# Autodesk Inventor assembly: Differential Swerve Drive V3
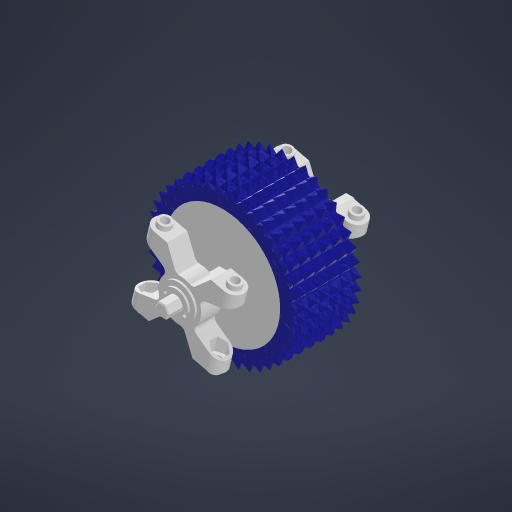
[picture p0: Inventor's stored thumbnail of the model, 512x512]
Saved by Autodesk Inventor 2024 (Build 280153000, 153)
## iProperties
Created: 2023-09-09
Part Number: Differential Swerve Drive V3
Document SubType Name: Assembly
Designer: izack
Author: izack
## Documents named in this file (7)
- C:\Users\izack\Robotics\CAD\Custom-Modules-CAD\Differential Swerve Drive V1\Differential Swerve Drive V3.iam
- C:\Users\izack\Robotics\CAD\Custom-Modules-CAD\Differential Swerve Drive V1\Differential Swerve Drive V3\60mm Wheel Rim.ipt
- C:\Users\izack\Robotics\CAD\Custom-Modules-CAD\Differential Swerve Drive V1\Differential Swerve Drive V3\60mm Wheel Tire Tread.ipt
- C:\Users\izack\Robotics\CAD\Custom-Modules-CAD\Differential Swerve Drive V1\Differential Swerve Drive V3\5mm x 55mm Hex Shaft.ipt
- C:\Users\izack\Robotics\CAD\Custom-Modules-CAD\Differential Swerve Drive V1\Differential Swerve Drive V3\Center_Bracket.ipt
- C:\Users\izack\Robotics\CAD\Custom-Modules-CAD\Differential Swerve Drive V1\Differential Swerve Drive V3\Flanged_Bearing.ipt
- C:\Users\izack\Robotics\CAD\Custom-Modules-CAD\Differential Swerve Drive V1\Differential Swerve Drive V3\5mm Hex to 8mm Round Bearing Insert.ipt
## Components (13 placed, 6 different names)
1. 60mm Wheel Rim:1 — Flush:1, Mate:1, Mate:2
2. 60mm Wheel Tire Tread:1 — Flush:1
3. 5mm x 55mm Hex Shaft:1 — Mate:1, Mate:2, Mate:19, Mate:20, Mate:21, Mate:23, Mate:24
4. Center_Bracket:1 — Mate:5, Mate:6, Mate:13, Mate:14, Flush:2
5. Center_Bracket:2 — Mate:15, Mate:16, Mate:17, Mate:18, Mate:22, Flush:2
6. Flanged_Bearing:1 — Mate:11, Mate:12, Mate:17, Mate:18
7. Flanged_Bearing:2 — Mate:9, Mate:10, Mate:15, Mate:16, Mate:22
8. Flanged_Bearing:3 — Mate:3, Mate:4, Mate:5, Mate:6
9. Flanged_Bearing:4 — Mate:7, Mate:8, Mate:13, Mate:14
10. 5mm Hex to 8mm Round Bearing Insert:1 — Mate:11, Mate:12, Mate:21, Mate:23
11. 5mm Hex to 8mm Round Bearing Insert:2 — Mate:9, Mate:10, Mate:24
12. 5mm Hex to 8mm Round Bearing Insert:3 — Mate:7, Mate:8
13. 5mm Hex to 8mm Round Bearing Insert:4 — Mate:3, Mate:4, Mate:19, Mate:20
## Relationships (26: Mate 24, Flush 2)
- Flush:1: 60mm Wheel Rim:1 ↔ 60mm Wheel Tire Tread:1
- Mate:1: 60mm Wheel Rim:1 ↔ 5mm x 55mm Hex Shaft:1
- Mate:2: 60mm Wheel Rim:1 ↔ 5mm x 55mm Hex Shaft:1
- Mate:3: Flanged_Bearing:3 ↔ 5mm Hex to 8mm Round Bearing Insert:4
- Mate:4: Flanged_Bearing:3 ↔ 5mm Hex to 8mm Round Bearing Insert:4
- Mate:5: Center_Bracket:1 ↔ Flanged_Bearing:3
- Mate:6: Center_Bracket:1 ↔ Flanged_Bearing:3
- Mate:7: Flanged_Bearing:4 ↔ 5mm Hex to 8mm Round Bearing Insert:3
- Mate:8: Flanged_Bearing:4 ↔ 5mm Hex to 8mm Round Bearing Insert:3
- Mate:9: Flanged_Bearing:2 ↔ 5mm Hex to 8mm Round Bearing Insert:2
- Mate:10: Flanged_Bearing:2 ↔ 5mm Hex to 8mm Round Bearing Insert:2
- Mate:11: Flanged_Bearing:1 ↔ 5mm Hex to 8mm Round Bearing Insert:1
- Mate:12: Flanged_Bearing:1 ↔ 5mm Hex to 8mm Round Bearing Insert:1
- Mate:13: Center_Bracket:1 ↔ Flanged_Bearing:4
- Mate:14: Center_Bracket:1 ↔ Flanged_Bearing:4
- Mate:15: Center_Bracket:2 ↔ Flanged_Bearing:2
- Mate:16: Center_Bracket:2 ↔ Flanged_Bearing:2
- Mate:17: Center_Bracket:2 ↔ Flanged_Bearing:1
- Mate:18: Center_Bracket:2 ↔ Flanged_Bearing:1
- Mate:19: 5mm x 55mm Hex Shaft:1 ↔ 5mm Hex to 8mm Round Bearing Insert:4
- Mate:20: 5mm x 55mm Hex Shaft:1 ↔ 5mm Hex to 8mm Round Bearing Insert:4
- Mate:21: 5mm x 55mm Hex Shaft:1 ↔ 5mm Hex to 8mm Round Bearing Insert:1
- Mate:22: Center_Bracket:2 ↔ Flanged_Bearing:2
- Mate:23: 5mm x 55mm Hex Shaft:1 ↔ 5mm Hex to 8mm Round Bearing Insert:1
- Mate:24: 5mm x 55mm Hex Shaft:1 ↔ 5mm Hex to 8mm Round Bearing Insert:2
- Flush:2: Center_Bracket:1 ↔ Center_Bracket:2
